# Autodesk Inventor assembly: Assembly1
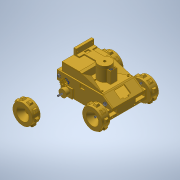
[picture p0: Inventor's stored thumbnail of the model, 180x180]
Saved by Autodesk Inventor 2020 (Build 240168000, 168)
## iProperties
Created: 2020-01-27
Part Number: Assembly1
Document SubType Name: Assembly
Designer: blep
Author: blep
## Documents named in this file (30)
- C:\Users\blep\Desktop\3d\scanning-robot\Assembly1.iam
- C:\Users\blep\Desktop\3d\scanning-robot\base.ipt
- C:\Users\blep\Desktop\3d\Tower Pro MG90S Micro servo\Tower Pro MG90S Micro servo.iam
- C:\Users\blep\Desktop\3d\scanning-robot\cover.ipt
- C:\Users\blep\Desktop\3d\scanning-robot\cover2.ipt
- C:\Users\blep\Desktop\3d\scanning-robot\arm.ipt
- C:\Users\blep\Documents\Inventor\Content Center Files\R2020\pl-PL\AS 1427(08)\AS 1427 - M4 x 16(6) I.ipt
- C:\Users\blep\Desktop\3d\scanning-robot\wheel.ipt
- C:\Users\blep\Desktop\3d\scanning-robot\wheel_MIR.ipt
- C:\Users\blep\Desktop\3d\scanning-robot\wheel_FRONT.ipt
- C:\Users\blep\Desktop\3d\scanning-robot\wheel_FRONT_MIR.ipt
- C:\Users\blep\Desktop\3d\scanning-robot\wheel-adapter.ipt
- C:\Users\blep\Desktop\3d\scanning-robot\wheel-adapter-front.ipt
- C:\Users\blep\Desktop\3d\scanning-robot\wheel-adapter-rear.ipt
- C:\Users\blep\Documents\Inventor\Content Center Files\R2020\pl-PL\AS 1112 (2)\AS 1112 - M4  Typ 5.ipt
- C:\Users\blep\Documents\Inventor\Content Center Files\R2020\pl-PL\AS 1237 (3.1)\AS 1237 - 4 mm(1)Aluminium-6061.ipt
- C:\Users\blep\Desktop\3d\scanning-robot\rod.ipt
- C:\Users\blep\Desktop\3d\scanning-robot\rod_CPY1.ipt
- C:\Users\blep\Desktop\3d\scanning-robot\rod_CPY2.ipt
- C:\Users\blep\Desktop\3d\scanning-robot\rod_CPY3.ipt
- C:\Users\blep\Desktop\3d\scanning-robot\wheel-adapter_MIR.ipt
- C:\Users\blep\Desktop\3d\scanning-robot\wheel-adapter-rear_MIR.ipt
- C:\Users\blep\Desktop\3d\scanning-robot\rod_MIR.ipt
- C:\Users\blep\Desktop\3d\scanning-robot\rod_CPY1_MIR.ipt
- C:\Users\blep\Desktop\3d\scanning-robot\rod_CPY2_MIR.ipt
- C:\Users\blep\Desktop\3d\scanning-robot\rod_CPY3_MIR.ipt
- C:\Users\blep\Desktop\3d\scanning-robot\coupler.ipt
- C:\Users\blep\Desktop\3d\scanning-robot\small-gear.ipt
- C:\Users\blep\Desktop\3d\scanning-robot\small-gear_MIR.ipt
- C:\Users\blep\Desktop\3d\scanning-robot\Assembly1\Design Accelerator\Przekładnie walcowe1.iam
## Components (60 placed, 29 different names)
1. Tower Pro MG90S Micro servo:1 [sub-assembly] — Mate:1, Mate:6, Mate:7, Obrotowe:27
2. Tower Pro MG90S Micro servo:2 [sub-assembly] — Mate:8, Mate:9, Mate:10, Obrotowe:26
3. base:1 — Mate:1, Mate:6, Mate:7, Mate:8, Mate:9, Mate:10, Rigid:1, Sztywne:4, Sztywne:5, Równoległe:1, Symetria:1, Sztywne:37, Sztywne:47
4. cover:1 — Rigid:1, Rigid:2, Rigid:3, Symetria:1
5. cover2:1 — Rigid:2
6. arm:1 — Rotational:15
7. wheel-adapter:1 — Równoległe:1, Sztywne:6, Obrotowe:16, Sztywne:7, Sztywne:12, Sztywne:18, Sztywne:19, Sztywne:20, Sztywne:21, Sztywne:47, Sztywne:48, Sztywne:50, Sztywne:55, Sztywne:56
8. wheel-adapter-front:1 — Sztywne:56, Sztywne:57, Sztywne:58, Sztywne:59, Sztywne:60, Obrotowe:30, Obrotowe:31
9. wheel-adapter-rear:1
10. wheel-adapter_MIR:1 — Sztywne:24, Obrotowe:17, Sztywne:26, Sztywne:29, Sztywne:33, Sztywne:34, Sztywne:35, Sztywne:36, Sztywne:37, Sztywne:45, Sztywne:49
11. wheel-adapter-rear_MIR:1 — Sztywne:25, Sztywne:52
12. coupler:1 — Sztywne:48, Sztywne:53, Sztywne:54
13. small-gear:1 — Obrotowe:26
14. small-gear_MIR:1 — Obrotowe:27
15. Przekładnie walcowe:1 [sub-assembly]
16. AS 1112 (2) - Metryczny M4  Typ 5:10 — Sztywne:55
17. wheel:1
18. wheel_MIR:1
19. wheel_FRONT:1 — Obrotowe:31
20. wheel_FRONT_MIR:1 — Obrotowe:30
21. AS 1427 Z - Metryczny M4 x 16:8 — Sztywne:59
22. AS 1427 Z - Metryczny M4 x 16:9 — Sztywne:60
23. AS 1427 Z - Metryczny M4 x 16:10
24. AS 1427 Z - Metryczny M4 x 16:11 — Sztywne:50
25. AS 1112 (2) - Metryczny M4  Typ 5:6 — Sztywne:54
26. AS 1112 (2) - Metryczny M4  Typ 5:7 — Sztywne:53
27. AS 1427 Z - Metryczny M4 x 16:12 — Sztywne:49
28. AS 1427 Z - Metryczny M4 x 16:13 — Sztywne:52
29. AS 1112 (2) - Metryczny M4  Typ 5:9 — Sztywne:45
30. AS 1237 (3.1) 4 mm - Aluminium 6061:12 — Sztywne:32
31. AS 1427 Z - Metryczny M4 x 16:6 — Sztywne:58
32. AS 1427 Z - Metryczny M4 x 16:7
33. AS 1112 (2) - Metryczny M4  Typ 5:4 — Sztywne:24
34. AS 1112 (2) - Metryczny M4  Typ 5:5 — Obrotowe:17
35. AS 1237 (3.1) 4 mm - Aluminium 6061:7 — Sztywne:25, Sztywne:27
36. AS 1237 (3.1) 4 mm - Aluminium 6061:8 — Sztywne:26, Sztywne:28
37. AS 1237 (3.1) 4 mm - Aluminium 6061:9 — Sztywne:27, Sztywne:28
38. AS 1237 (3.1) 4 mm - Aluminium 6061:10 — Sztywne:29, Sztywne:30
39. AS 1237 (3.1) 4 mm - Aluminium 6061:11 — Sztywne:30, Sztywne:32
40. AS 1427 Z - Metryczny M4 x 16:1 — Sztywne:4
41. AS 1427 Z - Metryczny M4 x 16:2 — Sztywne:5
42. AS 1427 Z - Metryczny M4 x 16:4 — Sztywne:57
43. AS 1427 Z - Metryczny M4 x 16:5
44. AS 1112 (2) - Metryczny M4  Typ 5:1 — Sztywne:6
45. AS 1112 (2) - Metryczny M4  Typ 5:3 — Obrotowe:16
46. AS 1237 (3.1) 4 mm - Aluminium 6061:1 — Sztywne:9
47. AS 1237 (3.1) 4 mm - Aluminium 6061:2 — Sztywne:7, Sztywne:8
48. AS 1237 (3.1) 4 mm - Aluminium 6061:3 — Sztywne:8, Sztywne:9
49. AS 1237 (3.1) 4 mm - Aluminium 6061:4 — Sztywne:12, Sztywne:13
50. AS 1237 (3.1) 4 mm - Aluminium 6061:6 — Sztywne:14
51. AS 1237 (3.1) 4 mm - Aluminium 6061:5 — Sztywne:13, Sztywne:14
52. rod_MIR:1 — Sztywne:33
53. rod_CPY1_MIR:1 — Sztywne:34
54. rod_CPY2_MIR:1 — Sztywne:35
55. rod_CPY3_MIR:1 — Sztywne:36
56. rod:1 — Sztywne:18
57. rod_CPY1:1 — Sztywne:19
58. rod_CPY2:1 — Sztywne:20
59. rod_CPY3:1 — Sztywne:21
60. Tower Pro MG90S Micro servo:3 [sub-assembly] — Rigid:3, Rotational:15
## Relationships (58: WeldJoint 43, RevoluteJoint 7, Mate 6, Flush 1, Symmetry 1)
- Mate:1: Tower Pro MG90S Micro servo:1 ↔ base:1
- Mate:6: Tower Pro MG90S Micro servo:1 ↔ base:1
- Mate:7: Tower Pro MG90S Micro servo:1 ↔ base:1
- Mate:8: Tower Pro MG90S Micro servo:2 ↔ base:1
- Mate:9: Tower Pro MG90S Micro servo:2 ↔ base:1
- Mate:10: Tower Pro MG90S Micro servo:2 ↔ base:1
- Rigid:1 [WeldJoint]: base:1 ↔ cover:1
- Rigid:2 [WeldJoint]: cover:1 ↔ cover2:1
- Rigid:3 [WeldJoint]: cover:1 ↔ Tower Pro MG90S Micro servo:3
- Rotational:15 [RevoluteJoint]: arm:1 ↔ Tower Pro MG90S Micro servo:3
- Sztywne:4 [WeldJoint]: base:1 ↔ AS 1427 Z - Metryczny M4 x 16:1
- Sztywne:5 [WeldJoint]: base:1 ↔ AS 1427 Z - Metryczny M4 x 16:2
- Równoległe:1 [Flush]: base:1 ↔ wheel-adapter:1
- Sztywne:6 [WeldJoint]: wheel-adapter:1 ↔ AS 1112 (2) - Metryczny M4  Typ 5:1
- Obrotowe:16 [RevoluteJoint]: wheel-adapter:1 ↔ AS 1112 (2) - Metryczny M4  Typ 5:3
- Sztywne:7 [WeldJoint]: wheel-adapter:1 ↔ AS 1237 (3.1) 4 mm - Aluminium 6061:2
- Sztywne:8 [WeldJoint]: AS 1237 (3.1) 4 mm - Aluminium 6061:2 ↔ AS 1237 (3.1) 4 mm - Aluminium 6061:3
- Sztywne:9 [WeldJoint]: AS 1237 (3.1) 4 mm - Aluminium 6061:1 ↔ AS 1237 (3.1) 4 mm - Aluminium 6061:3
- Sztywne:12 [WeldJoint]: wheel-adapter:1 ↔ AS 1237 (3.1) 4 mm - Aluminium 6061:4
- Sztywne:13 [WeldJoint]: AS 1237 (3.1) 4 mm - Aluminium 6061:4 ↔ AS 1237 (3.1) 4 mm - Aluminium 6061:5
- Sztywne:14 [WeldJoint]: AS 1237 (3.1) 4 mm - Aluminium 6061:6 ↔ AS 1237 (3.1) 4 mm - Aluminium 6061:5
- Sztywne:18 [WeldJoint] (-20 mm): wheel-adapter:1 ↔ rod:1
- Sztywne:19 [WeldJoint] (-20 mm): wheel-adapter:1 ↔ rod_CPY1:1
- Sztywne:20 [WeldJoint] (20 mm): wheel-adapter:1 ↔ rod_CPY2:1
- Sztywne:21 [WeldJoint] (-20 mm): wheel-adapter:1 ↔ rod_CPY3:1
- Symetria:1 [Symmetry]: base:1 ↔ cover:1
- Sztywne:24 [WeldJoint]: wheel-adapter_MIR:1 ↔ AS 1112 (2) - Metryczny M4  Typ 5:4
- Obrotowe:17 [RevoluteJoint]: wheel-adapter_MIR:1 ↔ AS 1112 (2) - Metryczny M4  Typ 5:5
- Sztywne:25 [WeldJoint]: wheel-adapter-rear_MIR:1 ↔ AS 1237 (3.1) 4 mm - Aluminium 6061:7
- Sztywne:26 [WeldJoint]: wheel-adapter_MIR:1 ↔ AS 1237 (3.1) 4 mm - Aluminium 6061:8
- Sztywne:27 [WeldJoint]: AS 1237 (3.1) 4 mm - Aluminium 6061:7 ↔ AS 1237 (3.1) 4 mm - Aluminium 6061:9
- Sztywne:28 [WeldJoint]: AS 1237 (3.1) 4 mm - Aluminium 6061:8 ↔ AS 1237 (3.1) 4 mm - Aluminium 6061:9
- Sztywne:29 [WeldJoint]: wheel-adapter_MIR:1 ↔ AS 1237 (3.1) 4 mm - Aluminium 6061:10
- Sztywne:30 [WeldJoint]: AS 1237 (3.1) 4 mm - Aluminium 6061:10 ↔ AS 1237 (3.1) 4 mm - Aluminium 6061:11
- Sztywne:32 [WeldJoint]: AS 1237 (3.1) 4 mm - Aluminium 6061:12 ↔ AS 1237 (3.1) 4 mm - Aluminium 6061:11
- Sztywne:33 [WeldJoint] (20 mm): wheel-adapter_MIR:1 ↔ rod_MIR:1
- Sztywne:34 [WeldJoint] (20 mm): wheel-adapter_MIR:1 ↔ rod_CPY1_MIR:1
- Sztywne:35 [WeldJoint] (20 mm): wheel-adapter_MIR:1 ↔ rod_CPY2_MIR:1
- Sztywne:36 [WeldJoint] (20 mm): wheel-adapter_MIR:1 ↔ rod_CPY3_MIR:1
- Sztywne:37 [WeldJoint]: base:1 ↔ wheel-adapter_MIR:1
- Sztywne:45 [WeldJoint]: wheel-adapter_MIR:1 ↔ AS 1112 (2) - Metryczny M4  Typ 5:9
- Obrotowe:26 [RevoluteJoint]: Tower Pro MG90S Micro servo:2 ↔ small-gear:1
- Obrotowe:27 [RevoluteJoint]: Tower Pro MG90S Micro servo:1 ↔ small-gear_MIR:1
- Sztywne:47 [WeldJoint]: base:1 ↔ wheel-adapter:1
- Sztywne:48 [WeldJoint]: wheel-adapter:1 ↔ coupler:1
- Sztywne:49 [WeldJoint]: wheel-adapter_MIR:1 ↔ AS 1427 Z - Metryczny M4 x 16:12
- Sztywne:50 [WeldJoint]: wheel-adapter:1 ↔ AS 1427 Z - Metryczny M4 x 16:11
- Sztywne:52 [WeldJoint]: wheel-adapter-rear_MIR:1 ↔ AS 1427 Z - Metryczny M4 x 16:13
- Sztywne:53 [WeldJoint]: coupler:1 ↔ AS 1112 (2) - Metryczny M4  Typ 5:7
- Sztywne:54 [WeldJoint]: coupler:1 ↔ AS 1112 (2) - Metryczny M4  Typ 5:6
- Sztywne:55 [WeldJoint]: wheel-adapter:1 ↔ AS 1112 (2) - Metryczny M4  Typ 5:10
- Sztywne:56 [WeldJoint] (2.4 mm): wheel-adapter:1 ↔ wheel-adapter-front:1
- Sztywne:57 [WeldJoint]: wheel-adapter-front:1 ↔ AS 1427 Z - Metryczny M4 x 16:4
- Sztywne:58 [WeldJoint]: wheel-adapter-front:1 ↔ AS 1427 Z - Metryczny M4 x 16:6
- Sztywne:59 [WeldJoint]: wheel-adapter-front:1 ↔ AS 1427 Z - Metryczny M4 x 16:8
- Sztywne:60 [WeldJoint]: wheel-adapter-front:1 ↔ AS 1427 Z - Metryczny M4 x 16:9
- Obrotowe:30 [RevoluteJoint] (0.4 mm): wheel-adapter-front:1 ↔ wheel_FRONT_MIR:1
- Obrotowe:31 [RevoluteJoint] (0.4 mm): wheel-adapter-front:1 ↔ wheel_FRONT:1
